# Autodesk Inventor assembly: tip_plate
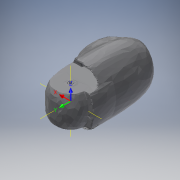
[picture p0: Inventor's stored thumbnail of the model, 180x180]
Saved by Autodesk Inventor 2019 (Build 230136000, 136)
## iProperties
Created: 2024-08-26
Part Number: tip_plate
Material: Generisch
Document SubType Name: Assembly
Designer: nic
Author: nic
## Documents named in this file (2)
- C:\Users\Nicolas Frick\Sync\OneDrive\wtm\nicol_rh8d\inventor\tip_plate.iam
- C:\Users\Nicolas Frick\Sync\OneDrive\wtm\nias\nias_description\inventor_files\hand\r_rh8d_refac\tip_refac.ipt
## Components (1 placed, 1 different names)
1. tip_refac:1 — Passend:1, Passend:2, Fluchtend:1
## Relationships (3: Mate 2, Flush 1)
- Passend:1 [Mate]: tip_refac:1
- Passend:2 [Mate]: tip_refac:1
- Fluchtend:1 [Flush]: tip_refac:1
